# Autodesk Inventor assembly: DriveChain2
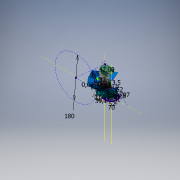
[picture p0: Inventor's stored thumbnail of the model, 180x180]
Saved by Autodesk Inventor 2018.3 (Build 223284000, 284)
## iProperties
Created: 2018-07-27
Part Number: DriveChain2
Material: Generisch
Document SubType Name: Assembly
Designer: JochenAlt
Author: JochenAlt
## Documents named in this file (12)
- D:\Projects\FlowerPot\CAD\DriveChain.iam
- D:\Projects\FlowerPot\CAD\Motor.iam
- D:\Projects\FlowerPot\CAD\HarmonicDrive-Axis.ipt
- D:\Projects\FlowerPot\CAD\BushOmniWheel.ipt
- D:\Projects\FlowerPot\CAD\OmniWheel-66mm.ipt
- D:\Projects\FlowerPot\CAD\Mounting Hub.ipt
- D:\Projects\FlowerPot\CAD\Encoder\Avago Encoder.iam
- D:\Projects\FlowerPot\CAD\DriveChainEnclosure2.ipt
- D:\Projects\FlowerPot\CAD\Spindle\SpindleThread.ipt
- D:\Projects\FlowerPot\CAD\Beltdrive\BeltDrive.iam
- D:\Projects\FlowerPot\CAD\AST_Bearings_SMR74ZZ.ipt
- C:\Users\JochenAlt\Documents\Inventor\Content Center Files\R2018\de-DE\SKF - Single row ball bearings\SKF623.ipt
## Components (12 placed, 11 different names)
1. Motor:1 [sub-assembly] — Passend:44, Passend:53, Passend:58, Passend:59, Passend:60
2. HarmonicDrive-Axis:1 — Passend:11, Passend:13, Drehung:4, Passend:15
3. BushOmniWheel:1 — Passend:11, Passend:14
4. OmniWheel:1 — Passend:15, Passend:16, Drehung:6
5. Mounting Hub:1 — Passend:13, Drehung:4, Passend:14, Passend:16, Drehung:6
6. Avago Encoder:1 [sub-assembly] — Passend:57, Passend:58, Passend:59
7. DriveChainEnclosure:1 — Passend:44, Passend:68, Passend:69, Passend:70
8. SpindleThread:1 — Passend:69, Passend:70
9. BeltDriveTest:1 [sub-assembly] — Passend:53, Passend:54, Passend:57, Passend:60
10. AST_Bearings_SMR74ZZ:1
11. AST_Bearings_SMR74ZZ:2
12. SKF- Kugellager, einreihig SKF623:1 — Passend:68
## Relationships (17: Mate 15, RelateRotation 2)
- Passend:11 [Mate]: HarmonicDrive-Axis:1 ↔ BushOmniWheel:1
- Passend:13 [Mate]: HarmonicDrive-Axis:1 ↔ Mounting Hub:1
- Drehung:4 [RelateRotation] (-1 ul): HarmonicDrive-Axis:1 ↔ Mounting Hub:1
- Passend:14 [Mate]: BushOmniWheel:1 ↔ Mounting Hub:1
- Passend:15 [Mate]: HarmonicDrive-Axis:1 ↔ OmniWheel:1
- Passend:16 [Mate]: OmniWheel:1 ↔ Mounting Hub:1
- Drehung:6 [RelateRotation] (1 ul): OmniWheel:1 ↔ Mounting Hub:1
- Passend:44 [Mate]: Motor:1 ↔ DriveChainEnclosure:1
- Passend:53 [Mate]: Motor:1 ↔ BeltDriveTest:1
- Passend:54 [Mate]: BeltDriveTest:1
- Passend:57 [Mate]: Avago Encoder:1 ↔ BeltDriveTest:1
- Passend:58 [Mate]: Motor:1 ↔ Avago Encoder:1
- Passend:59 [Mate] (0.5 mm): Motor:1 ↔ Avago Encoder:1
- Passend:60 [Mate] (0.5 mm): Motor:1 ↔ BeltDriveTest:1
- Passend:68 [Mate]: DriveChainEnclosure:1 ↔ SKF- Kugellager, einreihig SKF623:1
- Passend:69 [Mate]: DriveChainEnclosure:1 ↔ SpindleThread:1
- Passend:70 [Mate]: DriveChainEnclosure:1 ↔ SpindleThread:1
